# Autodesk Inventor assembly: Humidifier
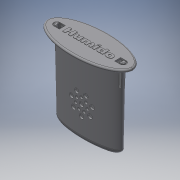
[picture p0: Inventor's stored thumbnail of the model, 180x180]
Saved by Autodesk Inventor 2016 (Build 200138000, 138)
## iProperties
Created: 2018-11-09
Part Number: Humidifier
Document SubType Name: Assembly
Designer: Justin
Author: Justin
## Documents named in this file (3)
- C:\Users\Justin\Documents\3D Design\Guitar Humidifier\Humidifier.iam
- C:\Users\Justin\Documents\3D Design\Guitar Humidifier\Top Lid.ipt
- C:\Users\Justin\Documents\3D Design\Guitar Humidifier\Part2.ipt
## Components (2 placed, 2 different names)
1. Top Lid:1 — Mate:1, Mate:3
2. Part2:1 — Mate:2, Mate:3
## Relationships (3: Mate 3)
- Mate:1: Top Lid:1
- Mate:2: Part2:1
- Mate:3: Top Lid:1 ↔ Part2:1
